# Autodesk Inventor assembly: Shoulder_horn_frame_WearingImage
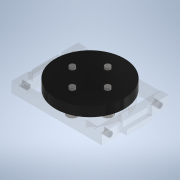
[picture p0: Inventor's stored thumbnail of the model, 180x180]
Saved by Autodesk Inventor 2020.4 (Build 244396000, 396)
## iProperties
Created: 2022-03-16
Part Number: Shoulder_horn_frame_WearingImage
Document SubType Name: Assembly
Designer: Masato Kubotera
Author: Masato Kubotera
## Documents named in this file (4)
- C:\Users\Masato\Documents\Inventor\CIT Brains_Inventor\SUSTAINA-OP\SandBlastingJig\Shoulder_horn_frame_WearingImage.iam
- C:\Users\Masato\Documents\Inventor\CIT Brains_Inventor\SUSTAINA-OP\SandBlastingJig\Shoulder_horn_frame_SandBlastingJig.ipt
- C:\Users\Masato\Documents\Inventor\CIT Brains_Inventor\SUSTAINA-OP\UpperBody\Arm\Shoulder_horn_frame.ipt
- C:\Users\Masato\Documents\Inventor\CIT Brains_Inventor\SUSTAINA-OP\ReadyMade\Screw\M2_6-10.ipt
## Components (6 placed, 3 different names)
1. Shoulder_horn_frame_SandBlastingJig:1 — 挿入:1
2. Shoulder_horn_frame:1 — 挿入:1, 挿入:2, 挿入:3, 挿入:4, 挿入:5
3. M2_6-10:1 — 挿入:5
4. M2_6-10:2 — 挿入:4
5. M2_6-10:3 — 挿入:3
6. M2_6-10:4 — 挿入:2
## Relationships (5: Insert 5)
- 挿入:1 [Insert]: Shoulder_horn_frame_SandBlastingJig:1 ↔ Shoulder_horn_frame:1
- 挿入:2 [Insert]: Shoulder_horn_frame:1 ↔ M2_6-10:4
- 挿入:3 [Insert]: Shoulder_horn_frame:1 ↔ M2_6-10:3
- 挿入:4 [Insert]: Shoulder_horn_frame:1 ↔ M2_6-10:2
- 挿入:5 [Insert]: Shoulder_horn_frame:1 ↔ M2_6-10:1
